# Autodesk Inventor assembly: ASY GnG station
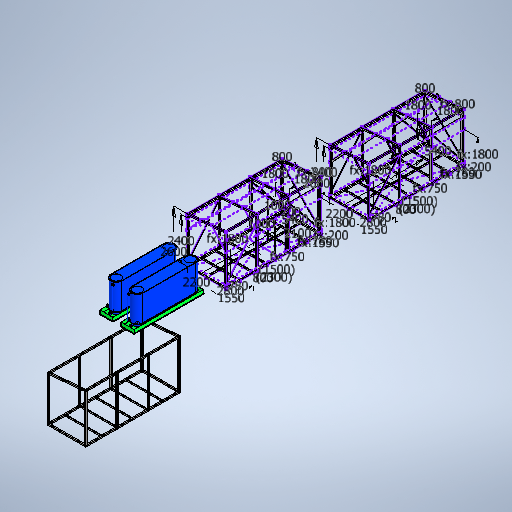
[picture p0: Inventor's stored thumbnail of the model, 512x512]
Saved by Autodesk Inventor 2025 (Build 290162010, 162A)
## iProperties
Created: 2025-09-20
Part Number: ASY GnG station
Document SubType Name: Assembly
Designer: admin
Mass: 766899 g
Surface Area: 646346 cm^2
Volume: 96834.3 cm^3
Density: 7.91971 g/cm^3
Author: admin
## Documents named in this file (7)
- C:\Users\admin\Yandex.Disk\home pc\Inventor\GnG_Gantul_hill\ASY GnG station.iam
- C:\Users\admin\Yandex.Disk\home pc\Inventor\GnG_Gantul_hill\GNG НаOCl pan.ipt
- C:\Users\admin\Yandex.Disk\home pc\Inventor\GnG_Gantul_hill\GNG НаOCl tank 2.ipt
- C:\Users\admin\Yandex.Disk\home pc\Inventor\GnG_Gantul_hill\GNG НаOCl tank 2_MIR.ipt
- C:\Users\admin\Yandex.Disk\home pc\Inventor\GnG_Gantul_hill\ASY GnG frame 1.iam
- C:\Users\admin\Yandex.Disk\home pc\Inventor\GnG_Gantul_hill\ASY GnG frame 2.iam
- C:\Users\admin\Yandex.Disk\home pc\Inventor\GnG_Gantul_hill\ASY GnG frame 1.1.iam
## Components (7 placed, 6 different names)
1. GNG НаOCl pan:1 — Mate:6, Flush:2, Tangent:1, Mate:9, Rigid:1
2. GNG НаOCl pan:2 — Flush:2, Rigid:1
3. GNG НаOCl tank 2:1 — Mate:6, Tangent:1, Mate:9, Rigid:2
4. GNG НаOCl tank 2_MIR:1 — Rigid:2
5. ASY GnG frame 1:1 [sub-assembly]
6. ASY GnG frame 2:1 [sub-assembly]
7. ASY GnG frame 1.1:1 [sub-assembly]
## Relationships (6: Mate 2, WeldJoint 2, Flush 1, Tangent 1)
- Mate:6 (40 mm): GNG НаOCl pan:1 ↔ GNG НаOCl tank 2:1
- Flush:2: GNG НаOCl pan:1 ↔ GNG НаOCl pan:2
- Tangent:1 (50 mm): GNG НаOCl pan:1 ↔ GNG НаOCl tank 2:1
- Mate:9: GNG НаOCl pan:1 ↔ GNG НаOCl tank 2:1
- Rigid:1 [WeldJoint] (400 mm): GNG НаOCl pan:1 ↔ GNG НаOCl pan:2
- Rigid:2 [WeldJoint] (600 mm): GNG НаOCl tank 2:1 ↔ GNG НаOCl tank 2_MIR:1
